# Autodesk Inventor assembly: .375'' Screw & Nylock Nut (Custom)
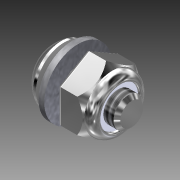
[picture p0: Inventor's stored thumbnail of the model, 180x180]
Saved by Autodesk Inventor 2012 (Build 160160000, 160)
## iProperties
Created: 2011-09-11
Part Number: .375'' Screw & Nylock Nut (Custom)
Document SubType Name: Assembly
Designer: Wade
Author: Wade
## Documents named in this file (4)
- C:\Users\Wade\Documents\1103 Robot - CAD Assembly\.375'' Screw & Nylock Nut (Custom).iam
- C:\Users\Wade\Documents\24C VEX CAD Files\Screws & Nuts\Screw 8-32 x 0.375''-Silver.ipt
- C:\Users\Wade\Documents\24C VEX CAD Files\Screws & Nuts\Nut 8-32 Nylock.ipt
- C:\Users\Wade\Documents\24C VEX CAD Files\Washers & Spacers\Washer, Steel.ipt
## Components (3 placed, 3 different names)
1. Screw 8-32 x 0.375''-Silver:1 — Mate:1, Mate:2, Mate:4
2. Nut 8-32 Nylock:1 — Mate:1, Mate:2, Mate:3
3. Washer, Steel:1 — Mate:3, Mate:4
## Relationships (4: Mate 4)
- Mate:1: Screw 8-32 x 0.375''-Silver:1 ↔ Nut 8-32 Nylock:1
- Mate:2 (3.1496 mm): Screw 8-32 x 0.375''-Silver:1 ↔ Nut 8-32 Nylock:1
- Mate:3 (1.1684 mm): Nut 8-32 Nylock:1 ↔ Washer, Steel:1
- Mate:4: Screw 8-32 x 0.375''-Silver:1 ↔ Washer, Steel:1
